# Autodesk Inventor assembly: 2 od flex with versa
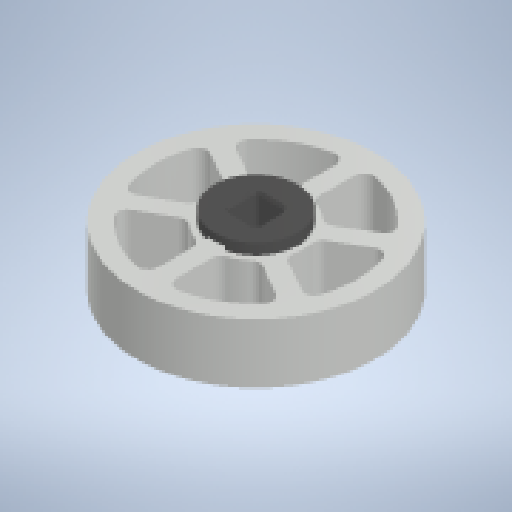
[picture p0: Inventor's stored thumbnail of the model, 512x512]
Saved by Autodesk Inventor 2023 (Build 270158000, 158)
## iProperties
Created: 2022-10-30
Part Number: 2 od flex with versa
Document SubType Name: Assembly
Designer: aaron
Author: aaron
## Documents named in this file (3)
- C:\Users\aaron\Documents\Inventor\Spin Up\library\Motion\Flex Wheels\2 od flex with versa.iam
- C:\Users\aaron\Documents\Inventor\Spin Up\library\Motion\Flex Wheels\2.0 OD flex.ipt
- C:\Users\aaron\Documents\Inventor\Spin Up\library\Motion\Flex Wheels\small versa.ipt
## Components (3 placed, 2 different names)
1. 2.0 OD flex:1 — Mate:1, Mate:2, Mate:3
2. small versa:1 — Flush:1, Flush:2, Mate:3
3. small versa:2 — Flush:1, Flush:2, Mate:1, Mate:2
## Relationships (5: Mate 3, Flush 2)
- Flush:1: small versa:1 ↔ small versa:2
- Flush:2: small versa:1 ↔ small versa:2
- Mate:1: 2.0 OD flex:1 ↔ small versa:2
- Mate:2: 2.0 OD flex:1 ↔ small versa:2
- Mate:3: 2.0 OD flex:1 ↔ small versa:1
